# Autodesk Inventor assembly: shaft_assembled
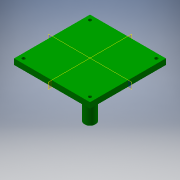
[picture p0: Inventor's stored thumbnail of the model, 180x180]
Saved by Autodesk Inventor 2016 (Build 200138000, 138)
## iProperties
Created: 2016-07-29
Part Number: shaft_assembled
Document SubType Name: Assembly
Designer: Fred
Author: Fred
## Documents named in this file (4)
- E:\DOCUMENTS\ROBOCUP-AT-WORK\MODELS\ARENA\ELEMENTS\DEVICES\ROTATING_TURNTABLE\INVENTOR\rotating_table_shaft_supported_assembly.iam
- E:\DOCUMENTS\ROBOCUP-AT-WORK\MODELS\ARENA\ELEMENTS\DEVICES\ROTATING_TURNTABLE\INVENTOR\rotating_table_shaft_plate.ipt
- E:\DOCUMENTS\ROBOCUP-AT-WORK\MODELS\ARENA\ELEMENTS\DEVICES\ROTATING_TURNTABLE\INVENTOR\rotating_table_shaft.ipt
- E:\documents\robocup-at-work\models\arena\elements\devices\rotating_turntable\inventor\rotating_table_shaft_strut.ipt
## Components (3 placed, 3 different names)
1. rotating_table_shaft_plate:1 — Mate:1, Mate:2, Mate:3, Flush:1
2. rotating_table_shaft:1 — Mate:1, Mate:2, Mate:3
3. rotating_table_shaft_strut:1 — Flush:1
## Relationships (4: Mate 3, Flush 1)
- Mate:1: rotating_table_shaft_plate:1 ↔ rotating_table_shaft:1
- Mate:2: rotating_table_shaft_plate:1 ↔ rotating_table_shaft:1
- Mate:3: rotating_table_shaft_plate:1 ↔ rotating_table_shaft:1
- Flush:1: rotating_table_shaft_plate:1 ↔ rotating_table_shaft_strut:1
